# Autodesk Inventor assembly: Left Angle Structure
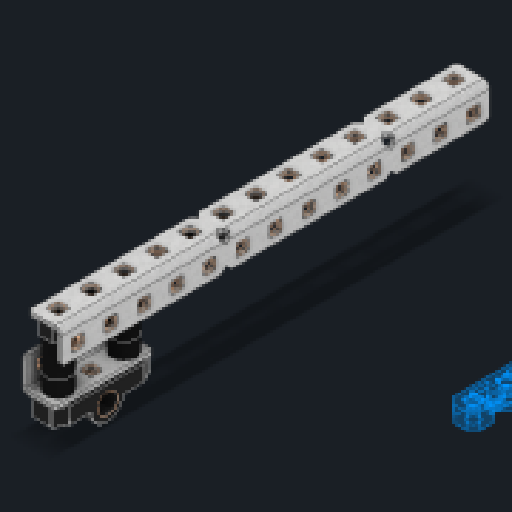
[picture p0: Inventor's stored thumbnail of the model, 512x512]
Saved by Autodesk Inventor 2025.1 (Build 291241000, 241)
## iProperties
Created: 2024-10-21
Part Number: Left Angle Structure
Document SubType Name: Assembly
Designer: averey
Author: averey
## Documents named in this file (10)
- C:\Users\avere\VEX\High Stakes\CAD\V3\Intake\Floating Stage\Left Angle Structure.iam
- C:\Users\avere\VEX\High Stakes\CAD\ROBOPROS-CAD-Inventor\Structure\Angle\Aluminum 1x1\Alu Angle 1x1x13.ipt
- C:\Users\avere\VEX\High Stakes\CAD\ROBOPROS-CAD-Inventor\Structure\Angle\Aluminum 1x1\Alu Angle 1x1x3.ipt
- C:\Users\avere\VEX\High Stakes\CAD\ROBOPROS-CAD-Inventor\Motion\Spacers\Spacer Nylon .375 OD\NSpacer .375 OD x .250.ipt
- C:\Users\avere\VEX\High Stakes\CAD\ROBOPROS-CAD-Inventor\Motion\Spacers\Spacer Nylon .375 OD.ipt
- C:\Users\avere\VEX\High Stakes\CAD\ROBOPROS-CAD-Inventor\Motion\Spacers\Spacer Nylon .375 OD\NSpacer .375 OD x .500.ipt
- C:\Users\avere\VEX\High Stakes\CAD\ROBOPROS-CAD-Inventor\Motion\Shaft HS\HS Pillow Bearing Block.ipt
- C:\Users\avere\VEX\High Stakes\CAD\ROBOPROS-CAD-Inventor\Structure\Hardware\Nut Nylon\Nut Nylon - White.ipt
- C:\Users\avere\VEX\High Stakes\CAD\ROBOPROS-CAD-Inventor\Structure\Hardware\Nut Nylon.ipt
- C:\Users\avere\VEX\High Stakes\CAD\ROBOPROS-CAD-Inventor\Motion\Shaft LS\Bearing Flat.ipt
## Components (11 placed, 7 different names)
1. Alu Angle 1x1x13:1 — Mate:1, Flush:1, Flush:2, Insert:3, Insert:6, Insert:10, Mate:3, Insert:11, Mate:4
2. Alu Angle 1x1x3:1 — Insert:4, Insert:7, Mate:2
3. NSpacer .375 OD x .250:1 — Insert:1
4. NSpacer .375 OD x .500:2 — Insert:1, Insert:3
5. NSpacer .375 OD x .250:3 — Insert:2, Insert:4
6. NSpacer .375 OD x .500:4 — Insert:2, Insert:6
7. HS Pillow Bearing Block:1 — Insert:7, Mate:2, Insert:8, Insert:9
8. Nut Nylon - White:1 — Insert:8
9. Nut Nylon - White:2 — Insert:9
10. Bearing Flat:1 — Insert:10, Mate:3
11. Bearing Flat:2 — Insert:11, Mate:4
## Relationships (16: Insert 10, Mate 4, Flush 2)
- Mate:1 (-82.55 mm): Alu Angle 1x1x13:1
- Flush:1: Alu Angle 1x1x13:1
- Flush:2: Alu Angle 1x1x13:1
- Insert:1: NSpacer .375 OD x .250:1 ↔ NSpacer .375 OD x .500:2
- Insert:2: NSpacer .375 OD x .250:3 ↔ NSpacer .375 OD x .500:4
- Insert:3 (6.35 mm): Alu Angle 1x1x13:1 ↔ NSpacer .375 OD x .500:2
- Insert:4: Alu Angle 1x1x3:1 ↔ NSpacer .375 OD x .250:3
- Insert:6 (6.35 mm): Alu Angle 1x1x13:1 ↔ NSpacer .375 OD x .500:4
- Insert:7: Alu Angle 1x1x3:1 ↔ HS Pillow Bearing Block:1
- Mate:2: Alu Angle 1x1x3:1 ↔ HS Pillow Bearing Block:1
- Insert:8: HS Pillow Bearing Block:1 ↔ Nut Nylon - White:1
- Insert:9: HS Pillow Bearing Block:1 ↔ Nut Nylon - White:2
- Insert:10: Alu Angle 1x1x13:1 ↔ Bearing Flat:1
- Mate:3: Alu Angle 1x1x13:1 ↔ Bearing Flat:1
- Insert:11: Alu Angle 1x1x13:1 ↔ Bearing Flat:2
- Mate:4: Alu Angle 1x1x13:1 ↔ Bearing Flat:2
